# Autodesk Inventor assembly: ServoHolder
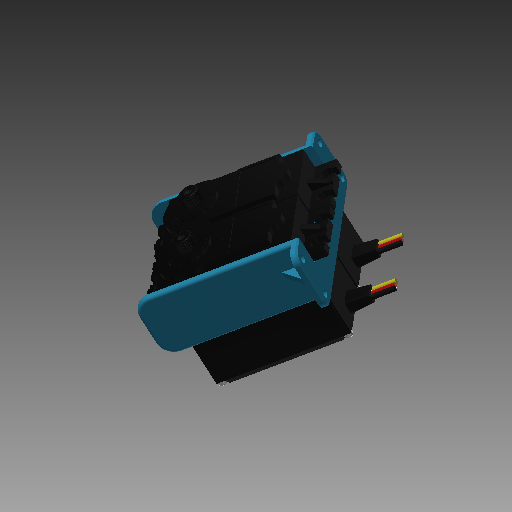
[picture p0: Inventor's stored thumbnail of the model, 512x512]
Saved by Autodesk Inventor 2018.2 (Build 222227000, 227)
## iProperties
Created: 2018-02-17
Part Number: ServoHolder
Material: Generisch
Document SubType Name: Assembly
Designer: JochenAlt
Author: JochenAlt
## Documents named in this file (3)
- D:\Projects\PrivateDancer\CAD\Servo-Holder.iam
- D:\Projects\PrivateDancer\CAD\hitec-hs-645mg\HS-645 MG.ipt
- D:\Projects\PrivateDancer\CAD\Stewart-Servo-Holder.ipt
## Components (3 placed, 2 different names)
1. HS-645 MG:1 — Passend:3, Passend:9, Passend:17
2. HS-645 MG:2 — Passend:1, Passend:8, Passend:16
3. Stewart-Servo-Holder:1 — Passend:1, Passend:3, Passend:8, Passend:9, Passend:16, Passend:17
## Relationships (6: Mate 6)
- Passend:1 [Mate] (0.3 mm): HS-645 MG:2 ↔ Stewart-Servo-Holder:1
- Passend:3 [Mate] (0.3 mm): HS-645 MG:1 ↔ Stewart-Servo-Holder:1
- Passend:8 [Mate] (0.3 mm): HS-645 MG:2 ↔ Stewart-Servo-Holder:1
- Passend:9 [Mate] (0.3 mm): HS-645 MG:1 ↔ Stewart-Servo-Holder:1
- Passend:16 [Mate] (0.3 mm): HS-645 MG:2 ↔ Stewart-Servo-Holder:1
- Passend:17 [Mate] (0.3 mm): HS-645 MG:1 ↔ Stewart-Servo-Holder:1
